# Autodesk Inventor assembly: linkage_system_test
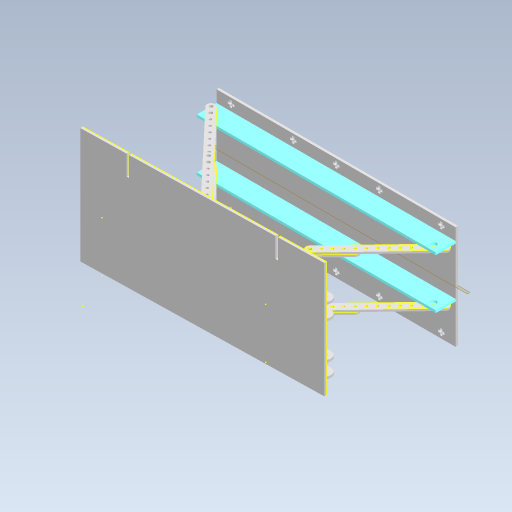
[picture p0: Inventor's stored thumbnail of the model, 512x512]
Saved by Autodesk Inventor 2023 (Build 270158000, 158)
## iProperties
Created: 2023-05-05
Part Number: linkage_system_test
Document SubType Name: Assembly
Designer: 陳詩穎
Author: 陳詩穎
## Documents named in this file (6)
- C:\Users\Johnny Jou\Documents\GitHub\Areo_Rider_Cabin\Expansion\test\linkage_system_test.iam
- C:\Users\Johnny Jou\Documents\GitHub\Areo_Rider_Cabin\Expansion\test\plate_expansion.ipt
- C:\Users\Johnny Jou\Documents\GitHub\Areo_Rider_Cabin\Expansion\test\零件1.ipt
- C:\Users\Johnny Jou\Documents\GitHub\Areo_Rider_Cabin\Expansion\test\adjustable.ipt
- C:\Users\Johnny Jou\Documents\GitHub\Areo_Rider_Cabin\Expansion\test\零件4.ipt
- C:\Users\Johnny Jou\Documents\GitHub\Areo_Rider_Cabin\Expansion\test\零件5.ipt
## Components (16 placed, 5 different names)
1. plate_expansion:1 — 貼合:1, 齊平:1, 貼合:2, 齊平:2, 齊平:6, 貼合:13
2. 零件1:1 — 齊平:2, 插入:1, 插入:4, 齊平:6, 貼合:13
3. 零件1:2 — 貼合:1, 齊平:1, 貼合:2, 插入:7, 插入:10
4. adjustable:1 — 插入:1, 插入:2, 插入:3
5. adjustable:2 — 插入:4, 插入:5, 插入:6
6. adjustable:3 — 插入:2, 插入:3, 相切:2, 貼合:6
7. adjustable:4 — 插入:5, 插入:6, 相切:1, 貼合:5
8. adjustable:5 — 插入:8, 插入:9, 相切:3, 貼合:7
9. adjustable:6 — 插入:10, 插入:11, 插入:12
10. adjustable:7 — 插入:11, 插入:12, 相切:4, 貼合:8
11. adjustable:8 — 插入:7, 插入:8, 插入:9
12. 零件4:1 — 相切:1, 貼合:5, 齊平:5, 貼合:11
13. 零件4:2 — 相切:2, 貼合:6, 齊平:4, 齊平:5, 貼合:10, 貼合:11
14. 零件4:3 — 相切:3, 貼合:7, 齊平:3, 齊平:4, 貼合:9, 貼合:10
15. 零件4:4 — 相切:4, 貼合:8, 齊平:3, 貼合:9, 貼合:14, 齊平:7, 貼合:15
16. 零件5:1 — 貼合:14, 齊平:7, 貼合:15
## Relationships (35: Mate 12, Insert 12, Flush 7, Tangent 4)
- 貼合:1 [Mate]: plate_expansion:1 ↔ 零件1:2
- 齊平:1 [Flush]: plate_expansion:1 ↔ 零件1:2
- 貼合:2 [Mate]: plate_expansion:1 ↔ 零件1:2
- 齊平:2 [Flush]: plate_expansion:1 ↔ 零件1:1
- 插入:1 [Insert]: 零件1:1 ↔ adjustable:1
- 插入:2 [Insert]: adjustable:1 ↔ adjustable:3
- 插入:3 [Insert]: adjustable:1 ↔ adjustable:3
- 插入:4 [Insert]: 零件1:1 ↔ adjustable:2
- 插入:5 [Insert]: adjustable:2 ↔ adjustable:4
- 插入:6 [Insert]: adjustable:2 ↔ adjustable:4
- 插入:7 [Insert]: 零件1:2 ↔ adjustable:8
- 插入:8 [Insert]: adjustable:5 ↔ adjustable:8
- 插入:9 [Insert]: adjustable:5 ↔ adjustable:8
- 插入:10 [Insert]: 零件1:2 ↔ adjustable:6
- 插入:11 [Insert]: adjustable:6 ↔ adjustable:7
- 插入:12 [Insert]: adjustable:6 ↔ adjustable:7
- 相切:1 [Tangent]: adjustable:4 ↔ 零件4:1
- 貼合:5 [Mate]: adjustable:4 ↔ 零件4:1
- 相切:2 [Tangent]: adjustable:3 ↔ 零件4:2
- 貼合:6 [Mate]: adjustable:3 ↔ 零件4:2
- 相切:3 [Tangent]: adjustable:5 ↔ 零件4:3
- 貼合:7 [Mate]: adjustable:5 ↔ 零件4:3
- 相切:4 [Tangent]: adjustable:7 ↔ 零件4:4
- 貼合:8 [Mate]: adjustable:7 ↔ 零件4:4
- 齊平:3 [Flush]: 零件4:3 ↔ 零件4:4
- 齊平:4 [Flush]: 零件4:2 ↔ 零件4:3
- 齊平:5 [Flush]: 零件4:1 ↔ 零件4:2
- 貼合:9 [Mate]: 零件4:3 ↔ 零件4:4
- 貼合:10 [Mate]: 零件4:2 ↔ 零件4:3
- 貼合:11 [Mate]: 零件4:1 ↔ 零件4:2
- 齊平:6 [Flush]: plate_expansion:1 ↔ 零件1:1
- 貼合:13 [Mate]: plate_expansion:1 ↔ 零件1:1
- 貼合:14 [Mate]: 零件4:4 ↔ 零件5:1
- 齊平:7 [Flush]: 零件4:4 ↔ 零件5:1
- 貼合:15 [Mate]: 零件4:4 ↔ 零件5:1
